# Autodesk Inventor assembly: StoveTopAssembly.ipt
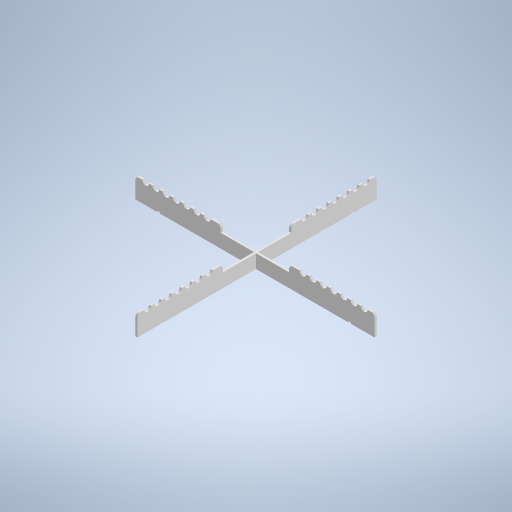
[picture p0: Inventor's stored thumbnail of the model, 512x512]
Saved by Autodesk Inventor 2024.3 (Build 283343000, 343)
## iProperties
Created: 2025-08-09
Part Number: StoveTopAssembly.ipt
Document SubType Name: Assembly
Designer: ajclo
Author: ajclo
## Documents named in this file (3)
- C:\Users\ajclo\OneDrive - Stellenbosch University\Documents\BEng\Year IV\Skripsie\CAD\CAD Final Design\StoveTopAssembly.ipt.iam
- C:\Users\ajclo\OneDrive - Stellenbosch University\Documents\BEng\Year IV\Skripsie\CAD\CAD Final Design\StoveTop2.ipt
- C:\Users\ajclo\OneDrive - Stellenbosch University\Documents\BEng\Year IV\Skripsie\CAD\CAD Final Design\StoveTop1.ipt
## Components (2 placed, 2 different names)
1. StoveTop2:1 — Mate:1, Mate:2, Mate:3
2. StoveTop1:1 — Mate:1, Mate:2, Mate:3
## Relationships (3: Mate 3)
- Mate:1: StoveTop2:1 ↔ StoveTop1:1
- Mate:2 (0.05 mm): StoveTop2:1 ↔ StoveTop1:1
- Mate:3 (0.05 mm): StoveTop2:1 ↔ StoveTop1:1
